# Autodesk Inventor assembly: new_u64_shoulder
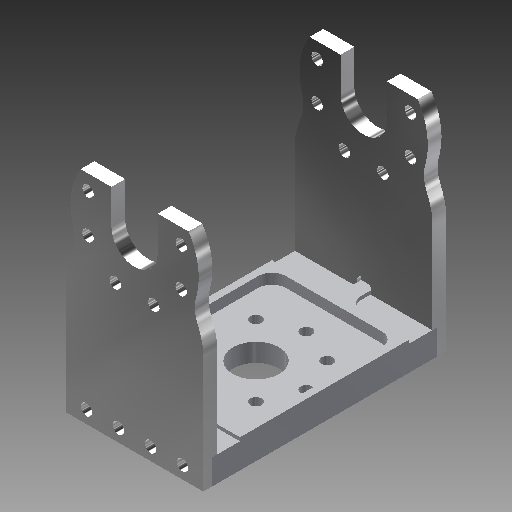
[picture p0: Inventor's stored thumbnail of the model, 512x512]
Saved by Autodesk Inventor 2018 (Build 220112000, 112)
## iProperties
Created: 2017-05-18
Part Number: new_u64_shoulder
Document SubType Name: Assembly
Designer: steve
Mass: 23.6618 g
Surface Area: 103.412 cm^2
Volume: 12.3361 cm^3
Density: 1.91809 g/cm^3
Author: steve
## Documents named in this file (3)
- C:\Users\etd\Dropbox\SigmaBan\SigmaBanV2.1\new_u64_shoulder.iam
- C:\Users\etd\Dropbox\SigmaBan\SigmaBanV2.1\new_base_u64_long.ipt
- C:\Users\etd\Dropbox\SigmaBan\SigmaBanV2.1\test_side_u64.ipt
## Components (3 placed, 2 different names)
1. new_base_u64_long:1 — Mate:1, Mate:2, Mate:3, Mate:4, Mate:5, Mate:6
2. test_side_u64:1 — Mate:1, Mate:2, Mate:3
3. test_side_u64:2 — Mate:4, Mate:5, Mate:6
## Relationships (6: Mate 6)
- Mate:1: new_base_u64_long:1 ↔ test_side_u64:1
- Mate:2: new_base_u64_long:1 ↔ test_side_u64:1
- Mate:3: new_base_u64_long:1 ↔ test_side_u64:1
- Mate:4: new_base_u64_long:1 ↔ test_side_u64:2
- Mate:5: new_base_u64_long:1 ↔ test_side_u64:2
- Mate:6: new_base_u64_long:1 ↔ test_side_u64:2
